# Autodesk Inventor assembly: 42146-25
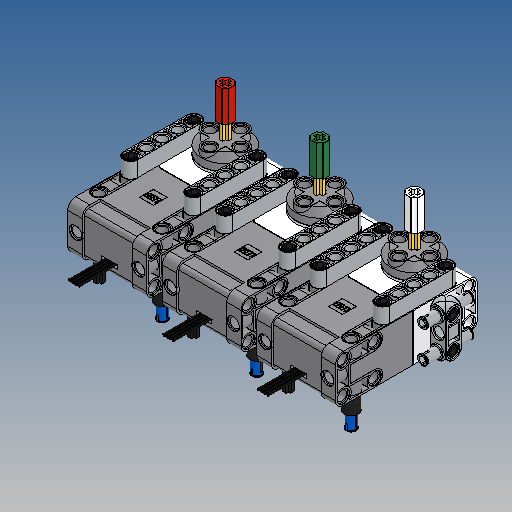
[picture p0: Inventor's stored thumbnail of the model, 512x512]
Saved by Autodesk Inventor 2025 (Build 290162010, 162A)
## iProperties
Created: 2024-11-24
Part Number: 42146-25
Material: Generisch
Document SubType Name: Assembly
Designer: hp.muther
Author: hp.muther
## Documents named in this file (12)
- D:\Inventor\Projekte\Muther\LEGO Technic\LEGO Technik - Raupenkran LR 13000 (42146)\42146-25.iam
- D:\Inventor\Projekte\Muther\LEGO Technic\LEGO Pieces\69730 - MOTOR, NR. 15.ipt
- D:\Inventor\Projekte\Muther\LEGO Technic\LEGO Pieces\Pin's\2780-Black.ipt
- D:\Inventor\Projekte\Muther\LEGO Technic\LEGO Pieces\Lochbalken\32316-LtBluishGray.ipt
- D:\Inventor\Projekte\Muther\LEGO Technic\LEGO Pieces\Verbindungselemente\48989-LtBluishGray.ipt
- D:\Inventor\Projekte\Muther\LEGO Technic\LEGO Pieces\Rund\6538c-White.ipt
- D:\Inventor\Projekte\Muther\LEGO Technic\LEGO Pieces\Rund\6538c-Green.ipt
- D:\Inventor\Projekte\Muther\LEGO Technic\LEGO Pieces\Rund\6538c-Red.ipt
- D:\Inventor\Projekte\Muther\LEGO Technic\LEGO Pieces\Achsen\4519-Yellow.ipt
- D:\Inventor\Projekte\Muther\LEGO Technic\LEGO Pieces\Rund\18654-Black.ipt
- D:\Inventor\Projekte\Muther\LEGO Technic\LEGO Pieces\Pin's\6558-Blue.ipt
- D:\Inventor\Projekte\Muther\LEGO Technic\LEGO Pieces\Pin's\18651-Black.ipt
## Components (42 placed, 11 different names)
1. 69730 - MOTOR, NR. 15:1 — Einfügen:5, Einfügen:6, Passend:1, Passend:2, Einfügen:7, Einfügen:11, Einfügen:13, Einfügen:38, Passend:8, Einfügen:40, Passend:9
2. 2780-Black:1 — Einfügen:1
3. 2780-Black:2 — Einfügen:2, Passend:1
4. 32316-LtBluishGray:1 — Einfügen:1, Einfügen:2, Einfügen:6
5. 2780-Black:3 — Passend:2
6. 2780-Black:4
7. 32316-LtBluishGray:2 — Einfügen:5
8. 2780-Black:5 — Einfügen:10, Passend:8
9. 2780-Black:6 — Einfügen:9
10. 48989-LtBluishGray:1 — Einfügen:9, Einfügen:10, Einfügen:38
11. 6538c-White:1 — Einfügen:8
12. 4519-Yellow:1 — Einfügen:7, Einfügen:8
13. 18654-Black:1 — Einfügen:12
14. 6558-Blue:1 — Einfügen:12, Einfügen:13
15. 18651-Black:1 — Einfügen:11
16. 69730 - MOTOR, NR. 15:2 — Einfügen:40, Einfügen:41, Passend:9, Passend:10
17. 2780-Black:7
18. 2780-Black:8
19. 32316-LtBluishGray:3
20. 2780-Black:9
21. 2780-Black:10
22. 32316-LtBluishGray:4
23. 6538c-Green:1
24. 4519-Yellow:2
25. 18654-Black:2
26. 6558-Blue:2
27. 18651-Black:2
28. 69730 - MOTOR, NR. 15:3 — Einfügen:39, Passend:7, Einfügen:41, Passend:10
29. 2780-Black:11
30. 2780-Black:12
31. 32316-LtBluishGray:5
32. 2780-Black:13
33. 2780-Black:14
34. 32316-LtBluishGray:6
35. 6538c-Red:1
36. 4519-Yellow:3
37. 18654-Black:3
38. 6558-Blue:3
39. 18651-Black:3
40. 2780-Black:15
41. 2780-Black:16 — Passend:7
42. 48989-LtBluishGray:2 — Einfügen:39
## Relationships (51: Insert 41, Mate 10)
- Einfügen:1 [Insert]: 2780-Black:1 ↔ 32316-LtBluishGray:1
- Einfügen:2 [Insert]: 2780-Black:2 ↔ 32316-LtBluishGray:1
- [Insert]: 2780-Black:3 ↔ 32316-LtBluishGray:2
- [Insert]: 2780-Black:4 ↔ 32316-LtBluishGray:2
- Einfügen:5 [Insert]: 69730 - MOTOR, NR. 15:1 ↔ 32316-LtBluishGray:2
- Einfügen:6 [Insert]: 69730 - MOTOR, NR. 15:1 ↔ 32316-LtBluishGray:1
- Passend:1 [Mate]: 69730 - MOTOR, NR. 15:1 ↔ 2780-Black:2
- Passend:2 [Mate]: 69730 - MOTOR, NR. 15:1 ↔ 2780-Black:3
- Einfügen:7 [Insert] (-8 mm): 69730 - MOTOR, NR. 15:1 ↔ 4519-Yellow:1
- Einfügen:8 [Insert] (-8 mm): 6538c-White:1 ↔ 4519-Yellow:1
- Einfügen:9 [Insert]: 2780-Black:6 ↔ 48989-LtBluishGray:1
- Einfügen:10 [Insert]: 2780-Black:5 ↔ 48989-LtBluishGray:1
- Einfügen:11 [Insert]: 69730 - MOTOR, NR. 15:1 ↔ 18651-Black:1
- Einfügen:12 [Insert]: 18654-Black:1 ↔ 6558-Blue:1
- Einfügen:13 [Insert]: 69730 - MOTOR, NR. 15:1 ↔ 6558-Blue:1
- [Insert]: 2780-Black:7 ↔ 32316-LtBluishGray:3
- [Insert]: 2780-Black:8 ↔ 32316-LtBluishGray:3
- [Insert]: 2780-Black:9 ↔ 32316-LtBluishGray:4
- [Insert]: 2780-Black:10 ↔ 32316-LtBluishGray:4
- [Insert]: 69730 - MOTOR, NR. 15:2 ↔ 32316-LtBluishGray:4
- [Insert]: 69730 - MOTOR, NR. 15:2 ↔ 32316-LtBluishGray:3
- [Mate]: 69730 - MOTOR, NR. 15:2 ↔ 2780-Black:8
- [Mate]: 69730 - MOTOR, NR. 15:2 ↔ 2780-Black:9
- [Insert] (-8 mm): 69730 - MOTOR, NR. 15:2 ↔ 4519-Yellow:2
- [Insert] (-8 mm): 6538c-Green:1 ↔ 4519-Yellow:2
- [Insert]: 69730 - MOTOR, NR. 15:2 ↔ 18651-Black:2
- [Insert]: 18654-Black:2 ↔ 6558-Blue:2
- [Insert]: 69730 - MOTOR, NR. 15:2 ↔ 6558-Blue:2
- [Insert]: 2780-Black:11 ↔ 32316-LtBluishGray:5
- [Insert]: 2780-Black:12 ↔ 32316-LtBluishGray:5
- [Insert]: 2780-Black:13 ↔ 32316-LtBluishGray:6
- [Insert]: 2780-Black:14 ↔ 32316-LtBluishGray:6
- [Insert]: 69730 - MOTOR, NR. 15:3 ↔ 32316-LtBluishGray:6
- [Insert]: 69730 - MOTOR, NR. 15:3 ↔ 32316-LtBluishGray:5
- [Mate]: 69730 - MOTOR, NR. 15:3 ↔ 2780-Black:12
- [Mate]: 69730 - MOTOR, NR. 15:3 ↔ 2780-Black:13
- [Insert] (-8 mm): 69730 - MOTOR, NR. 15:3 ↔ 4519-Yellow:3
- [Insert] (-8 mm): 6538c-Red:1 ↔ 4519-Yellow:3
- [Insert]: 69730 - MOTOR, NR. 15:3 ↔ 18651-Black:3
- [Insert]: 18654-Black:3 ↔ 6558-Blue:3
- [Insert]: 69730 - MOTOR, NR. 15:3 ↔ 6558-Blue:3
- [Insert]: 2780-Black:16 ↔ 48989-LtBluishGray:2
- [Insert]: 2780-Black:15 ↔ 48989-LtBluishGray:2
- Einfügen:38 [Insert]: 69730 - MOTOR, NR. 15:1 ↔ 48989-LtBluishGray:1
- Einfügen:39 [Insert]: 69730 - MOTOR, NR. 15:3 ↔ 48989-LtBluishGray:2
- Passend:7 [Mate]: 69730 - MOTOR, NR. 15:3 ↔ 2780-Black:16
- Passend:8 [Mate]: 69730 - MOTOR, NR. 15:1 ↔ 2780-Black:5
- Einfügen:40 [Insert] (8 mm): 69730 - MOTOR, NR. 15:1 ↔ 69730 - MOTOR, NR. 15:2
- Einfügen:41 [Insert] (8 mm): 69730 - MOTOR, NR. 15:2 ↔ 69730 - MOTOR, NR. 15:3
- Passend:9 [Mate]: 69730 - MOTOR, NR. 15:1 ↔ 69730 - MOTOR, NR. 15:2
- Passend:10 [Mate]: 69730 - MOTOR, NR. 15:2 ↔ 69730 - MOTOR, NR. 15:3
## Named parameters: d2_d0 = 0 mm, d3_d1 = 0 mm, d15_d0 = 0 mm, d16_d1 = 0 mm, d17_d2_d0 = 0 mm, d18_d3_d1 = 0 mm, d19_d4 = 0 mm, d20_d5 = 0 mm, d21_d6 = 0 mm, d22_d7 = 0 mm, d23_d8 = -8 mm, d24_d9 = -8 mm, d25_d12 = 0 mm, d26_d13 = 0 mm, d27_d14 = 0 mm, d28_d0 = 0 mm, d29_d1 = 0 mm, d30_d2_d0 = 0 mm, d31_d3_d1 = 0 mm, d32_d4 = 0 mm, d33_d5 = 0 mm, d34_d6 = 0 mm, d35_d7 = 0 mm, d36_d8 = -8 mm, d37_d9 = -8 mm, d38_d12 = 0 mm, d39_d13 = 0 mm, d40_d14 = 0 mm, d41_d10 = 0 mm, d42_d11 = 0 mm
